# Autodesk Inventor assembly: bloc_moteur
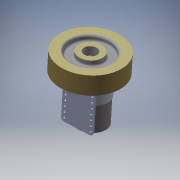
[picture p0: Inventor's stored thumbnail of the model, 180x180]
Saved by Autodesk Inventor 2017 (Build 210142000, 142)
## iProperties
Created: 2017-12-17
Part Number: bloc_moteur
Document SubType Name: Assembly
Designer: franc
Author: franc
## Documents named in this file (5)
- C:\Users\franc\Desktop\EsialRobotik\Mecanique\base_roulante\bloc_moteur.iam
- C:\Users\franc\Desktop\EsialRobotik\Mecanique\base_roulante\composants\37d-gearmotor-19-30.ipt
- C:\Users\franc\Desktop\EsialRobotik\Mecanique\base_roulante\composants\support_moteur.ipt
- C:\Users\franc\Desktop\EsialRobotik\Mecanique\base_roulante\composants\moyeu_serrage_conique.ipt
- C:\Users\franc\Desktop\EsialRobotik\Mecanique\base_roulante\composants\Colson_Wheel_3in_x_7_8in.ipt
## Components (4 placed, 4 different names)
1. 37d-gearmotor-19-30:1
2. support_moteur:1
3. moyeu_serrage_conique:1
4. Colson_Wheel_3in_x_7_8in:1
## Relationships (7: Mate 6, Flush 1)
- [Mate]: 37d-gearmotor-19-30:1 ↔ support_moteur:1
- [Mate]: 37d-gearmotor-19-30:1 ↔ moyeu_serrage_conique:1
- [Mate]: 37d-gearmotor-19-30:1 ↔ moyeu_serrage_conique:1
- [Mate]: moyeu_serrage_conique:1 ↔ Colson_Wheel_3in_x_7_8in:1
- [Flush]: moyeu_serrage_conique:1 ↔ Colson_Wheel_3in_x_7_8in:1
- [Mate]: 37d-gearmotor-19-30:1 ↔ support_moteur:1
- [Mate] (0.003 mm): 37d-gearmotor-19-30:1 ↔ support_moteur:1
## Named parameters: d16_d9 = 0 mm, d17_d11 = 0 mm, d18_d12 = 0 mm, d19_d13 = 0 mm, d20_d14 = 0 mm, d21_d1 = 0 mm
